# Autodesk Inventor assembly: ASY стапель
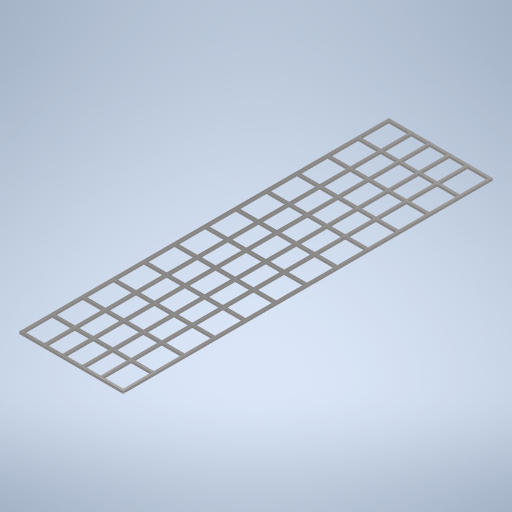
[picture p0: Inventor's stored thumbnail of the model, 512x512]
Saved by Autodesk Inventor 2024.2 (Build 282272000, 272)
## iProperties
Created: 2024-06-13
Part Number: ASY стапель
Document SubType Name: Assembly
Designer: admin
_SolveAssemblyDoc: Frame Generator Solve Assembly
_Version: 25.0.0
Author: admin
## Documents named in this file (3)
- C:\Users\admin\YandexDisk-badmisterfox\домашниий пк\Inventor\Manturovo\Manturovo_Se-clar\стапель\ASY стапель.iam
- C:\Users\admin\YandexDisk-badmisterfox\домашниий пк\Inventor\Manturovo\Manturovo_Se-clar\стапель\Эскиз стапель.ipt
- C:\Users\admin\YandexDisk-badmisterfox\домашниий пк\Inventor\Manturovo\Manturovo_Se-clar\стапель\ASY стапель\Frame\Frame 1718297263236.iam
## Components (2 placed, 2 different names)
1. Эскиз стапель:1 — Mate:1, Mate:2, Flush:1
2. Frame 1718297263236:1 [sub-assembly]
## Relationships (3: Mate 2, Flush 1)
- Mate:1: Эскиз стапель:1
- Mate:2: Эскиз стапель:1
- Flush:1: Эскиз стапель:1
